# Autodesk Inventor assembly: BG_Rumpf_Stecksystem_V
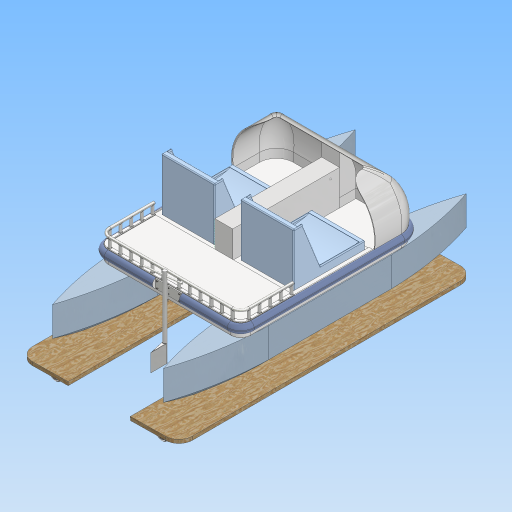
[picture p0: Inventor's stored thumbnail of the model, 512x512]
Saved by Autodesk Inventor 2024.4 (Build 284460000, 460)
## iProperties
Created: 2026-01-18
Part Number: BG_Rumpf_Stecksystem_V
Document SubType Name: Assembly
Designer: windows-desktop
Mass: 1.08187e+06 g
Surface Area: 662359 cm^2
Volume: 926557 cm^3
Density: 1.16762 g/cm^3
Author: windows-desktop
## Documents named in this file (12)
- C:\Users\windows-desktop\Desktop\Studium\Konstruktion\VaultWorkspace\Daten\I60-Konstruktion\I60-Gruppe-4\Bluhm\Daten\I60-Konstruktion\I60-Gruppe-4\Bluhm\Gesamt_Konstruktion\BG_Rumpf_Stecksystem.iam
- C:\Users\windows-desktop\Desktop\Studium\Konstruktion\VaultWorkspace\Daten\I60-Konstruktion\I60-Gruppe-4\Bluhm\Daten\I60-Konstruktion\I60-Gruppe-4\Bluhm\Deck\Verbindungsstück_Rumpf_Stecksystem.ipt
- C:\Users\windows-desktop\Desktop\Studium\Konstruktion\VaultWorkspace\Daten\I60-Konstruktion\I60-Gruppe-4\Bluhm\Daten\I60-Konstruktion\I60-Gruppe-4\Bluhm\Rumpf\Außenrumpf_schnittig.ipt
- C:\Users\windows-desktop\Desktop\Studium\Konstruktion\VaultWorkspace\Daten\I60-Konstruktion\I60-Gruppe-4\Bluhm\Daten\I60-Konstruktion\I60-Gruppe-4\Bluhm\Schrauben_Strang.ipt
- C:\Users\windows-desktop\Desktop\Studium\Konstruktion\VaultWorkspace\Daten\I60-Konstruktion\I60-Gruppe-4\Bluhm\Daten\I60-Konstruktion\I60-Gruppe-4\Bluhm\Deck_Getriebe\BG_Mittelkonsole.iam
- C:\Users\windows-desktop\Desktop\Studium\Konstruktion\VaultWorkspace\Daten\I60-Konstruktion\I60-Gruppe-4\Bluhm\Daten\I60-Konstruktion\I60-Gruppe-4\Bluhm\Antrieb\BG_Schiffschraube.iam
- C:\Users\windows-desktop\Desktop\Studium\Konstruktion\VaultWorkspace\Daten\I60-Konstruktion\I60-Gruppe-4\Bluhm\Daten\I60-Konstruktion\I60-Gruppe-4\Bluhm\Deck\Frontabdeckung.ipt
- C:\Users\windows-desktop\Desktop\Studium\Konstruktion\VaultWorkspace\Daten\I60-Konstruktion\I60-Gruppe-4\Bluhm\Daten\I60-Konstruktion\I60-Gruppe-4\Bluhm\Deck\Geländer.ipt
- C:\Users\windows-desktop\Desktop\Studium\Konstruktion\VaultWorkspace\Daten\I60-Konstruktion\I60-Gruppe-4\Bluhm\Daten\I60-Konstruktion\I60-Gruppe-4\Bluhm\Sitz\Sitz.ipt
- C:\Users\windows-desktop\Desktop\Studium\Konstruktion\VaultWorkspace\Daten\I60-Konstruktion\I60-Gruppe-4\Bluhm\Normteile\de-DE\ISO 4762(1)\DIN EN ISO 4762 - M10 x 16.ipt
- C:\Users\windows-desktop\Desktop\Studium\Konstruktion\VaultWorkspace\Daten\I60-Konstruktion\I60-Gruppe-4\Bluhm\Daten\I60-Konstruktion\I60-Gruppe-4\Bluhm\Transport\BG_Mattenwagen.iam
- C:\Users\windows-desktop\Desktop\Studium\Konstruktion\VaultWorkspace\Daten\I60-Konstruktion\I60-Gruppe-4\Bluhm\Daten\I60-Konstruktion\I60-Gruppe-4\Bluhm\Ruder\BG_Ruder.iam
## Components (20 placed, 11 different names)
1. Verbindungsstück_Rumpf_Stecksystem:1 — Einfügen:1, Einfügen:2, Einfügen:3, Einfügen:4, Passend:1, Einfügen:5, Einfügen:6, Einfügen:7, Fluchtend:1, Passend:5, Fluchtend:2, Passend:6, Passend:7, Passend:8, Passend:9, Passend:10, Passend:11, Passend:22, Passend:24, Passend:26, Passend:28, Einfügen:8, Einfügen:9, Passend:30, Passend:32, Passend:34, Passend:36
2. Außenrumpf_schnittig:1 — Einfügen:1, Einfügen:2
3. Außenrumpf_schnittig:2 — Einfügen:3, Einfügen:4
4. Schrauben_Strang:1 — Passend:1, Einfügen:5, Einfügen:6, Passend:2, Passend:3, Passend:4, Passend:23, Passend:25, Passend:27, Passend:29
5. BG_Mittelkonsole:1 [sub-assembly] — Einfügen:7
6. BG_Schiffschraube:1 [sub-assembly] — Passend:2, Passend:3, Passend:4
7. Frontabdeckung:1 — Fluchtend:1, Passend:5, Fluchtend:2
8. Geländer:1 — Passend:6, Passend:7
9. Sitz:1 — Passend:10, Passend:11
10. Sitz:2 — Passend:8, Passend:9
11. DIN EN ISO 4762 M10 x 16:5 — Passend:22, Passend:23
12. DIN EN ISO 4762 M10 x 16:6 — Passend:24, Passend:25
13. DIN EN ISO 4762 M10 x 16:7 — Passend:26, Passend:27
14. DIN EN ISO 4762 M10 x 16:8 — Passend:28, Passend:29
15. BG_Mattenwagen:1 [sub-assembly]
16. BG_Ruder:1 [sub-assembly] — Einfügen:8, Einfügen:9, Passend:31, Passend:33, Passend:35, Passend:37
17. DIN EN ISO 4762 M10 x 16:9 — Passend:30, Passend:31
18. DIN EN ISO 4762 M10 x 16:10 — Passend:32, Passend:33
19. DIN EN ISO 4762 M10 x 16:11 — Passend:34, Passend:35
20. DIN EN ISO 4762 M10 x 16:12 — Passend:36, Passend:37
## Relationships (38: Mate 27, Insert 9, Flush 2)
- Einfügen:1 [Insert]: Verbindungsstück_Rumpf_Stecksystem:1 ↔ Außenrumpf_schnittig:1
- Einfügen:2 [Insert]: Verbindungsstück_Rumpf_Stecksystem:1 ↔ Außenrumpf_schnittig:1
- Einfügen:3 [Insert]: Verbindungsstück_Rumpf_Stecksystem:1 ↔ Außenrumpf_schnittig:2
- Einfügen:4 [Insert]: Verbindungsstück_Rumpf_Stecksystem:1 ↔ Außenrumpf_schnittig:2
- Passend:1 [Mate]: Verbindungsstück_Rumpf_Stecksystem:1 ↔ Schrauben_Strang:1
- Einfügen:5 [Insert]: Verbindungsstück_Rumpf_Stecksystem:1 ↔ Schrauben_Strang:1
- Einfügen:6 [Insert]: Verbindungsstück_Rumpf_Stecksystem:1 ↔ Schrauben_Strang:1
- Passend:2 [Mate]: Schrauben_Strang:1 ↔ BG_Schiffschraube:1
- Passend:3 [Mate]: Schrauben_Strang:1 ↔ BG_Schiffschraube:1
- Einfügen:7 [Insert]: Verbindungsstück_Rumpf_Stecksystem:1 ↔ BG_Mittelkonsole:1
- Passend:4 [Mate]: Schrauben_Strang:1 ↔ BG_Schiffschraube:1
- Fluchtend:1 [Flush]: Verbindungsstück_Rumpf_Stecksystem:1 ↔ Frontabdeckung:1
- Passend:5 [Mate]: Verbindungsstück_Rumpf_Stecksystem:1 ↔ Frontabdeckung:1
- Fluchtend:2 [Flush]: Verbindungsstück_Rumpf_Stecksystem:1 ↔ Frontabdeckung:1
- Passend:6 [Mate]: Verbindungsstück_Rumpf_Stecksystem:1 ↔ Geländer:1
- Passend:7 [Mate]: Verbindungsstück_Rumpf_Stecksystem:1 ↔ Geländer:1
- Passend:8 [Mate]: Verbindungsstück_Rumpf_Stecksystem:1 ↔ Sitz:2
- Passend:9 [Mate]: Verbindungsstück_Rumpf_Stecksystem:1 ↔ Sitz:2
- Passend:10 [Mate]: Verbindungsstück_Rumpf_Stecksystem:1 ↔ Sitz:1
- Passend:11 [Mate]: Verbindungsstück_Rumpf_Stecksystem:1 ↔ Sitz:1
- Passend:22 [Mate]: Verbindungsstück_Rumpf_Stecksystem:1 ↔ DIN EN ISO 4762 M10 x 16:5
- Passend:23 [Mate]: Schrauben_Strang:1 ↔ DIN EN ISO 4762 M10 x 16:5
- Passend:24 [Mate]: Verbindungsstück_Rumpf_Stecksystem:1 ↔ DIN EN ISO 4762 M10 x 16:6
- Passend:25 [Mate]: Schrauben_Strang:1 ↔ DIN EN ISO 4762 M10 x 16:6
- Passend:26 [Mate]: Verbindungsstück_Rumpf_Stecksystem:1 ↔ DIN EN ISO 4762 M10 x 16:7
- Passend:27 [Mate]: Schrauben_Strang:1 ↔ DIN EN ISO 4762 M10 x 16:7
- Passend:28 [Mate]: Verbindungsstück_Rumpf_Stecksystem:1 ↔ DIN EN ISO 4762 M10 x 16:8
- Passend:29 [Mate]: Schrauben_Strang:1 ↔ DIN EN ISO 4762 M10 x 16:8
- Einfügen:8 [Insert]: Verbindungsstück_Rumpf_Stecksystem:1 ↔ BG_Ruder:1
- Einfügen:9 [Insert]: Verbindungsstück_Rumpf_Stecksystem:1 ↔ BG_Ruder:1
- Passend:30 [Mate]: Verbindungsstück_Rumpf_Stecksystem:1 ↔ DIN EN ISO 4762 M10 x 16:9
- Passend:31 [Mate]: BG_Ruder:1 ↔ DIN EN ISO 4762 M10 x 16:9
- Passend:32 [Mate]: Verbindungsstück_Rumpf_Stecksystem:1 ↔ DIN EN ISO 4762 M10 x 16:10
- Passend:33 [Mate]: BG_Ruder:1 ↔ DIN EN ISO 4762 M10 x 16:10
- Passend:34 [Mate]: Verbindungsstück_Rumpf_Stecksystem:1 ↔ DIN EN ISO 4762 M10 x 16:11
- Passend:35 [Mate]: BG_Ruder:1 ↔ DIN EN ISO 4762 M10 x 16:11
- Passend:36 [Mate]: Verbindungsstück_Rumpf_Stecksystem:1 ↔ DIN EN ISO 4762 M10 x 16:12
- Passend:37 [Mate]: BG_Ruder:1 ↔ DIN EN ISO 4762 M10 x 16:12
